# Autodesk Inventor assembly: hand
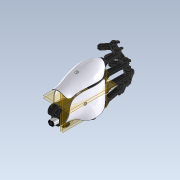
[picture p0: Inventor's stored thumbnail of the model, 180x180]
Saved by Autodesk Inventor 2020.2 (Build 242310000, 310)
## iProperties
Created: 2020-04-08
Part Number: hand
Document SubType Name: Assembly
Designer: Bardo91
thread_hole: 2.500 mm
Author: Bardo91
## Documents named in this file (25)
- D:\programming\elric\hardware\1. hand\elric20-01A.iam
- D:\programming\elric\hardware\1. hand\pinky_f1.ipt
- D:\programming\elric\hardware\1. hand\pinky_f2.ipt
- D:\programming\elric\hardware\1. hand\pinky_f3.ipt
- D:\programming\elric\hardware\1. hand\base_hand.ipt
- D:\programming\elric\hardware\1. hand\motor_dc_6v_30rpm.ipt
- D:\programming\elric\hardware\1. hand\finger_thread_lock.ipt
- D:\programming\elric\hardware\1. hand\finger_pulley.ipt
- D:\programming\elric\hardware\1. hand\ring_f2.ipt
- D:\programming\elric\hardware\1. hand\ring_f3.ipt
- D:\programming\elric\hardware\1. hand\ring_f1.ipt
- D:\programming\elric\hardware\1. hand\middle_f1.ipt
- D:\programming\elric\hardware\1. hand\middle_f2.ipt
- D:\programming\elric\hardware\1. hand\middle_f3.ipt
- D:\programming\elric\hardware\1. hand\index_f1.ipt
- D:\programming\elric\hardware\1. hand\index_f2.ipt
- D:\programming\elric\hardware\1. hand\index_f3.ipt
- D:\programming\elric\hardware\1. hand\thumb_f2.ipt
- D:\programming\elric\hardware\1. hand\thumb_f3.ipt
- D:\programming\elric\hardware\1. hand\thumb_f1.ipt
- D:\programming\elric\hardware\1. hand\cases\hand_case_1.ipt
- D:\programming\elric\hardware\1. hand\cases\hand_case_2.ipt
- D:\programming\elric\hardware\1. hand\cases\hand_case_3.ipt
- D:\programming\elric\hardware\1. hand\potentiometer_bourns_3382_12mm.ipt
- D:\programming\elric\hardware\1. hand\potentiometer_holder.ipt
## Components (39 placed, 24 different names)
1. base_hand:1 — Flush:9, Mate:12, Mate:32, Mate:33, Mate:36, Mate:37, Mate:40, Mate:41, Mate:78, Flush:18, Mate:79, Mate:80, Mate:81, Mate:83, Mate:84, Mate:85, Mate:87, Mate:88, Mate:89, Mate:92, Mate:93, Mate:94, Mate:95, Mate:96, Flush:19, Flush:20, Mate:98, Mate:99, Mate:100, Mate:102, Mate:103, Angle:1, Angle:2, Angle:3
2. hand_case_1:1
3. hand_case_2:1
4. hand_case_3:1
5. motor_dc_6v_30rpm:2 — Mate:105, Angle:1, Mate:106
6. potentiometer_holder:3 — Tangent:2, Mate:82, Mate:83, Mate:84, Mate:85, Mate:106
7. potentiometer_bourns_3382_12mm:6 — Tangent:2, Mate:82, Mate:105
8. finger_thread_lock:1 — Mate:25, Mate:26
9. pinky_f1:1 — Mate:1, Flush:1, Flush:9, Mate:12
10. pinky_f2:1 — Mate:1, Flush:1, Flush:2, Mate:2
11. pinky_f3:1 — Flush:2, Mate:2, Mate:25, Mate:26
12. motor_dc_6v_30rpm:1 — Mate:77, Mate:78, Flush:18
13. potentiometer_holder:1 — Mate:79, Mate:80, Mate:81, Tangent:1
14. potentiometer_bourns_3382_12mm:5 — Mate:77, Tangent:1
15. ring_f2:1 — Mate:30, Mate:31, Flush:10, Flush:11
16. ring_f3:1 — Mate:30, Flush:10
17. ring_f1:1 — Mate:31, Flush:11, Mate:32, Mate:33
18. potentiometer_holder:2 — Tangent:3, Mate:86, Mate:87, Mate:88, Mate:89, Mate:110
19. potentiometer_bourns_3382_12mm:3 — Tangent:3, Mate:86, Mate:109
20. motor_dc_6v_30rpm:4 — Angle:3, Mate:109, Mate:110
21. middle_f1:1 — Mate:35, Mate:36, Mate:37, Flush:12
22. middle_f2:1 — Mate:34, Mate:35, Flush:12, Flush:13
23. middle_f3:1 — Mate:34, Flush:13
24. potentiometer_bourns_3382_12mm:1 — Tangent:5, Mate:91, Mate:108
25. potentiometer_holder:5 — Tangent:5, Mate:91, Mate:92, Mate:93, Mate:94, Mate:107
26. motor_dc_6v_30rpm:3 — Mate:107, Mate:108, Angle:2
27. index_f1:1 — Mate:39, Mate:40, Flush:15, Mate:41
28. index_f2:1 — Mate:38, Mate:39, Flush:14, Flush:15
29. index_f3:1 — Mate:38, Flush:14
30. potentiometer_holder:6 — Tangent:6, Mate:101, Mate:102, Mate:103, Mate:104
31. potentiometer_holder:4 — Tangent:4, Mate:90, Mate:98, Mate:99, Mate:100
32. potentiometer_bourns_3382_12mm:4 — Tangent:6, Mate:101
33. potentiometer_bourns_3382_12mm:2 — Tangent:4, Mate:90
34. motor_dc_6v_30rpm:5 — Mate:95, Flush:19, Mate:97
35. motor_dc_6v_30rpm:6 — Mate:67, Mate:68, Mate:96, Flush:20, Mate:104
36. finger_pulley:5 — Mate:67, Mate:68
37. thumb_f1:1 — Mate:61, Flush:17, Mate:97
38. thumb_f2:1 — Mate:60, Mate:61, Flush:16, Flush:17
39. thumb_f3:1 — Mate:60, Flush:16
## Relationships (78: Mate 55, Flush 14, Tangent 6, Angle 3)
- Mate:1: pinky_f1:1 ↔ pinky_f2:1
- Flush:1: pinky_f1:1 ↔ pinky_f2:1
- Flush:2: pinky_f2:1 ↔ pinky_f3:1
- Mate:2: pinky_f2:1 ↔ pinky_f3:1
- Flush:9: base_hand:1 ↔ pinky_f1:1
- Mate:12: base_hand:1 ↔ pinky_f1:1
- Mate:25: finger_thread_lock:1 ↔ pinky_f3:1
- Mate:26 (0.25 mm): finger_thread_lock:1 ↔ pinky_f3:1
- Mate:30: ring_f2:1 ↔ ring_f3:1
- Mate:31: ring_f2:1 ↔ ring_f1:1
- Flush:10: ring_f2:1 ↔ ring_f3:1
- Flush:11: ring_f2:1 ↔ ring_f1:1
- Mate:32: base_hand:1 ↔ ring_f1:1
- Mate:33: base_hand:1 ↔ ring_f1:1
- Mate:34: middle_f2:1 ↔ middle_f3:1
- Mate:35: middle_f1:1 ↔ middle_f2:1
- Mate:36: base_hand:1 ↔ middle_f1:1
- Mate:37: base_hand:1 ↔ middle_f1:1
- Flush:12: middle_f1:1 ↔ middle_f2:1
- Flush:13: middle_f2:1 ↔ middle_f3:1
- Mate:38: index_f2:1 ↔ index_f3:1
- Mate:39: index_f1:1 ↔ index_f2:1
- Mate:40: base_hand:1 ↔ index_f1:1
- Flush:14: index_f2:1 ↔ index_f3:1
- Flush:15: index_f1:1 ↔ index_f2:1
- Mate:41: base_hand:1 ↔ index_f1:1
- Mate:60: thumb_f2:1 ↔ thumb_f3:1
- Mate:61: thumb_f1:1 ↔ thumb_f2:1
- Flush:16: thumb_f2:1 ↔ thumb_f3:1
- Flush:17: thumb_f1:1 ↔ thumb_f2:1
- Mate:67: motor_dc_6v_30rpm:6 ↔ finger_pulley:5
- Mate:68 (2.5 mm): motor_dc_6v_30rpm:6 ↔ finger_pulley:5
- Mate:77: motor_dc_6v_30rpm:1 ↔ potentiometer_bourns_3382_12mm:5
- Mate:78: base_hand:1 ↔ motor_dc_6v_30rpm:1
- Flush:18: base_hand:1 ↔ motor_dc_6v_30rpm:1
- Mate:79: base_hand:1 ↔ potentiometer_holder:1
- Mate:80: base_hand:1 ↔ potentiometer_holder:1
- Mate:81: base_hand:1 ↔ potentiometer_holder:1
- Tangent:1: potentiometer_holder:1 ↔ potentiometer_bourns_3382_12mm:5
- Tangent:2: potentiometer_holder:3 ↔ potentiometer_bourns_3382_12mm:6
- Mate:82: potentiometer_holder:3 ↔ potentiometer_bourns_3382_12mm:6
- Mate:83: base_hand:1 ↔ potentiometer_holder:3
- Mate:84: base_hand:1 ↔ potentiometer_holder:3
- Mate:85: base_hand:1 ↔ potentiometer_holder:3
- Tangent:3: potentiometer_holder:2 ↔ potentiometer_bourns_3382_12mm:3
- Mate:86: potentiometer_holder:2 ↔ potentiometer_bourns_3382_12mm:3
- Mate:87: base_hand:1 ↔ potentiometer_holder:2
- Mate:88: base_hand:1 ↔ potentiometer_holder:2
- Mate:89: base_hand:1 ↔ potentiometer_holder:2
- Tangent:4: potentiometer_holder:4 ↔ potentiometer_bourns_3382_12mm:2
- Tangent:5: potentiometer_bourns_3382_12mm:1 ↔ potentiometer_holder:5
- Mate:90: potentiometer_holder:4 ↔ potentiometer_bourns_3382_12mm:2
- Mate:91: potentiometer_bourns_3382_12mm:1 ↔ potentiometer_holder:5
- Mate:92: base_hand:1 ↔ potentiometer_holder:5
- Mate:93: base_hand:1 ↔ potentiometer_holder:5
- Mate:94: base_hand:1 ↔ potentiometer_holder:5
- Mate:95: base_hand:1 ↔ motor_dc_6v_30rpm:5
- Mate:96: base_hand:1 ↔ motor_dc_6v_30rpm:6
- Flush:19: base_hand:1 ↔ motor_dc_6v_30rpm:5
- Flush:20 (5 mm): base_hand:1 ↔ motor_dc_6v_30rpm:6
- Mate:97: motor_dc_6v_30rpm:5 ↔ thumb_f1:1
- Mate:98: base_hand:1 ↔ potentiometer_holder:4
- Mate:99: base_hand:1 ↔ potentiometer_holder:4
- Mate:100: base_hand:1 ↔ potentiometer_holder:4
- Tangent:6: potentiometer_holder:6 ↔ potentiometer_bourns_3382_12mm:4
- Mate:101: potentiometer_holder:6 ↔ potentiometer_bourns_3382_12mm:4
- Mate:102: base_hand:1 ↔ potentiometer_holder:6
- Mate:103: base_hand:1 ↔ potentiometer_holder:6
- Mate:104: potentiometer_holder:6 ↔ motor_dc_6v_30rpm:6
- Mate:105: motor_dc_6v_30rpm:2 ↔ potentiometer_bourns_3382_12mm:6
- Angle:1 (0 deg): base_hand:1 ↔ motor_dc_6v_30rpm:2
- Mate:106: motor_dc_6v_30rpm:2 ↔ potentiometer_holder:3
- Mate:107: potentiometer_holder:5 ↔ motor_dc_6v_30rpm:3
- Mate:108: potentiometer_bourns_3382_12mm:1 ↔ motor_dc_6v_30rpm:3
- Angle:2 (0 deg): base_hand:1 ↔ motor_dc_6v_30rpm:3
- Angle:3 (0 deg): base_hand:1 ↔ motor_dc_6v_30rpm:4
- Mate:109: potentiometer_bourns_3382_12mm:3 ↔ motor_dc_6v_30rpm:4
- Mate:110: potentiometer_holder:2 ↔ motor_dc_6v_30rpm:4
## Named parameters: thread_hole = 2.5 mm
